# Autodesk Inventor assembly: ElectronicsBayUpper
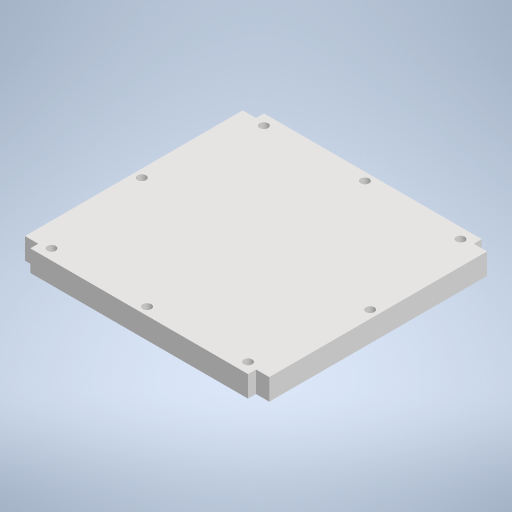
[picture p0: Inventor's stored thumbnail of the model, 512x512]
Saved by Autodesk Inventor 2023 (Build 270158000, 158)
## iProperties
Created: 2022-08-18
Part Number: ElectronicsBayUpper
Document SubType Name: Assembly
Designer: Aditya Bansal
Author: Aditya Bansal
## Documents named in this file (3)
- C:\Users\Aditya Bansal\OneDrive - UNSW\Uni\BlueSat\rocketry-datasat\Structure\Electronics_Structure\ElectronicsBayUpper.iam
- C:\Users\Aditya Bansal\OneDrive - UNSW\Uni\BlueSat\rocketry-datasat\Structure\Electronics_Structure\ElectronicsBayUpperMount.ipt
- C:\Users\Aditya Bansal\OneDrive - UNSW\Uni\BlueSat\rocketry-datasat\Structure\Electronics_Structure\DummyUpperBoard.ipt
## Components (2 placed, 2 different names)
1. ElectronicsBayUpperMount:1 — Mate:1, Mate:2
2. DummyUpperBoard:1 — Mate:1, Mate:2
## Relationships (2: Mate 2)
- Mate:1: ElectronicsBayUpperMount:1 ↔ DummyUpperBoard:1
- Mate:2: ElectronicsBayUpperMount:1 ↔ DummyUpperBoard:1
